# Autodesk Inventor assembly: КВ33.000.100 - Блок переключение передач
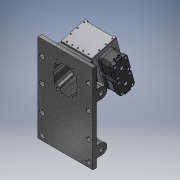
[picture p0: Inventor's stored thumbnail of the model, 180x180]
Saved by Autodesk Inventor 2019 (Build 230136000, 136)
## iProperties
Created: 2021-02-22
Part Number: КВ33.000.100 - Блок переключение передач
Material: Типовые
Document SubType Name: Assembly
Designer: Петров Иван
Author: Петров Иван
## Documents named in this file (12)
- E:\IVAN\Ivan_desktop\Kvantorium\Projects\tractor\design\КВ33.000.100 - Блок переключение передач.iam
- E:\IVAN\Ivan_desktop\Kvantorium\Projects\tractor\design\design_models\крышка КП.ipt
- E:\IVAN\Ivan_desktop\Kvantorium\Projects\tractor\design\КВ33.000.101 - Площадка крепежная.ipt
- E:\IVAN\Ivan_desktop\Kvantorium\Projects\tractor\design\КВ33.000.102 - Стенка толстая.ipt
- E:\IVAN\Ivan_desktop\Kvantorium\Projects\tractor\design\КВ33.000.103 - Стенка тонкая.ipt
- C:\Users\Петров Иван\Documents\Inventor\Content Center Files\R2019\en-US\GOST 9649-78\Washer 3 GOST 9649-78.ipt
- C:\Users\Петров Иван\Documents\Inventor\Content Center Files\R2019\en-US\Screw A2 GOST 17473-80\Screw A2.M2.5-6gx7 GOST 17473-80.ipt
- E:\IVAN\Ivan_desktop\Kvantorium\Projects\tractor\design\КВ33.000.104 - Крышка.ipt
- E:\IVAN\Ivan_desktop\Kvantorium\Projects\tractor\design\standart_components\Вал.ipt
- E:\IVAN\Ivan_desktop\Kvantorium\Projects\tractor\design\standart_components\Подшипник 626Z.ipt
- E:\IVAN\Ivan_desktop\Kvantorium\Projects\tractor\design\КВ33.000.105 - Заслонка.ipt
- E:\IVAN\Ivan_desktop\Kvantorium\Projects\tractor\design\standart_components\nema 17 motor.ipt
## Components (70 placed, 11 different names)
1. крышка КП:1 — Mate:1, Mate:8, Mate:9
2. КВ33.000.101 - Площадка крепежная:1 — Mate:1, Mate:3, Angle:1, Mate:4, Mate:6, Mate:8, Mate:9, Mate:21, Mate:27, Mate:28
3. КВ33.000.102 - Стенка толстая:1 — Mate:3, Angle:1, Insert:6, Insert:7, Insert:8, Insert:9, Insert:10, Mate:14, Mate:15, Mate:16, Mate:17, Mate:20, Mate:23, Angle:2, Angle:3, Mate:25, Mate:26
4. КВ33.000.102 - Стенка толстая:2 — Mate:4, Insert:1, Insert:2, Insert:3, Insert:4, Insert:5, Flush:4, Mate:10, Mate:11, Mate:12, Mate:13, Flush:5, Mate:28
5. КВ33.000.103 - Стенка тонкая:2 — Mate:6, Insert:22, Insert:23, Insert:24, Insert:25, Insert:26, Insert:27, Insert:28, Insert:29, Insert:30, Insert:31, Insert:32, Mate:21
6. КВ33.000.104 - Крышка:1 — Flush:4
7. Подшипник 626Z:1 — Mate:10, Mate:11, Mate:18
8. Подшипник 626Z:2 — Mate:14, Mate:15
9. Подшипник 626Z:3 — Mate:16, Mate:17
10. Подшипник 626Z:4 — Mate:12, Mate:13, Mate:19
11. Вал:1 — Mate:18, Flush:5, Flush:6, Mate:24
12. Вал:2 — Mate:19, Flush:6, Mate:22
13. КВ33.000.105 - Заслонка:1 — Mate:20
14. nema 17 motor:1 — Mate:22, Mate:23, Angle:2
15. nema 17 motor:2 — Mate:24, Angle:3
16. КВ33.000.103 - Стенка тонкая:3 — Mate:25, Mate:26, Mate:27
17. Washer GOST 9649-78 3:1 — Insert:1, Insert:49
18. Washer GOST 9649-78 3:2 — Insert:2, Insert:50
19. Washer GOST 9649-78 3:3 — Insert:3, Insert:51
20. Washer GOST 9649-78 3:4 — Insert:4, Insert:52
21. Washer GOST 9649-78 3:5 — Insert:5, Insert:53
22. Washer GOST 9649-78 3:6 — Insert:6, Insert:33
23. Washer GOST 9649-78 3:7 — Insert:7, Insert:34
24. Washer GOST 9649-78 3:8 — Insert:8, Insert:35
25. Washer GOST 9649-78 3:9 — Insert:9, Insert:36
26. Washer GOST 9649-78 3:10 — Insert:10, Insert:37
27. Washer GOST 9649-78 3:11 — Insert:42
28. Washer GOST 9649-78 3:12 — Insert:40
29. Washer GOST 9649-78 3:13 — Insert:41
30. Washer GOST 9649-78 3:14 — Insert:39
31. Washer GOST 9649-78 3:15 — Insert:38
32. Washer GOST 9649-78 3:16 — Insert:45
33. Washer GOST 9649-78 3:17 — Insert:44
34. Washer GOST 9649-78 3:18 — Insert:43
35. Washer GOST 9649-78 3:19 — Insert:46
36. Washer GOST 9649-78 3:20 — Insert:47
37. Washer GOST 9649-78 3:21 — Insert:48
38. Washer GOST 9649-78 3:22 — Insert:22
39. Washer GOST 9649-78 3:23 — Insert:23
40. Washer GOST 9649-78 3:24 — Insert:24
41. Washer GOST 9649-78 3:25 — Insert:25
42. Washer GOST 9649-78 3:26 — Insert:26
43. Washer GOST 9649-78 3:27 — Insert:27
44. Washer GOST 9649-78 3:28 — Insert:28
45. Washer GOST 9649-78 3:29 — Insert:29
46. Washer GOST 9649-78 3:30 — Insert:30, Insert:54
47. Washer GOST 9649-78 3:31 — Insert:31
48. Washer GOST 9649-78 3:32 — Insert:32
49. Screw A2 GOST 17473-80 M2.5-6gx7:1 — Insert:33
50. Screw A2 GOST 17473-80 M2.5-6gx7:2 — Insert:34
51. Screw A2 GOST 17473-80 M2.5-6gx7:3 — Insert:35
52. Screw A2 GOST 17473-80 M2.5-6gx7:4 — Insert:36
53. Screw A2 GOST 17473-80 M2.5-6gx7:5 — Insert:37
54. Screw A2 GOST 17473-80 M2.5-6gx7:6 — Insert:38
55. Screw A2 GOST 17473-80 M2.5-6gx7:7 — Insert:39
56. Screw A2 GOST 17473-80 M2.5-6gx7:8 — Insert:40
57. Screw A2 GOST 17473-80 M2.5-6gx7:9 — Insert:41
58. Screw A2 GOST 17473-80 M2.5-6gx7:10 — Insert:42
59. Screw A2 GOST 17473-80 M2.5-6gx7:11 — Insert:43
60. Screw A2 GOST 17473-80 M2.5-6gx7:12 — Insert:44
61. Screw A2 GOST 17473-80 M2.5-6gx7:13 — Insert:45
62. Screw A2 GOST 17473-80 M2.5-6gx7:14 — Insert:46
63. Screw A2 GOST 17473-80 M2.5-6gx7:15 — Insert:47
64. Screw A2 GOST 17473-80 M2.5-6gx7:16 — Insert:48
65. Screw A2 GOST 17473-80 M2.5-6gx7:17 — Insert:49
66. Screw A2 GOST 17473-80 M2.5-6gx7:18 — Insert:50
67. Screw A2 GOST 17473-80 M2.5-6gx7:19 — Insert:51
68. Screw A2 GOST 17473-80 M2.5-6gx7:20 — Insert:52
69. Screw A2 GOST 17473-80 M2.5-6gx7:21 — Insert:53
70. Screw A2 GOST 17473-80 M2.5-6gx7:22 — Insert:54
## Relationships (74: Insert 43, Mate 25, Angle 3, Flush 3)
- Mate:1: крышка КП:1 ↔ КВ33.000.101 - Площадка крепежная:1
- Mate:3: КВ33.000.101 - Площадка крепежная:1 ↔ КВ33.000.102 - Стенка толстая:1
- Angle:1 (0 deg): КВ33.000.101 - Площадка крепежная:1 ↔ КВ33.000.102 - Стенка толстая:1
- Mate:4: КВ33.000.101 - Площадка крепежная:1 ↔ КВ33.000.102 - Стенка толстая:2
- Mate:6: КВ33.000.101 - Площадка крепежная:1 ↔ КВ33.000.103 - Стенка тонкая:2
- Insert:1: КВ33.000.102 - Стенка толстая:2 ↔ Washer GOST 9649-78 3:1
- Insert:2: КВ33.000.102 - Стенка толстая:2 ↔ Washer GOST 9649-78 3:2
- Insert:3: КВ33.000.102 - Стенка толстая:2 ↔ Washer GOST 9649-78 3:3
- Insert:4: КВ33.000.102 - Стенка толстая:2 ↔ Washer GOST 9649-78 3:4
- Insert:5: КВ33.000.102 - Стенка толстая:2 ↔ Washer GOST 9649-78 3:5
- Insert:6: КВ33.000.102 - Стенка толстая:1 ↔ Washer GOST 9649-78 3:6
- Insert:7: КВ33.000.102 - Стенка толстая:1 ↔ Washer GOST 9649-78 3:7
- Insert:8: КВ33.000.102 - Стенка толстая:1 ↔ Washer GOST 9649-78 3:8
- Insert:9: КВ33.000.102 - Стенка толстая:1 ↔ Washer GOST 9649-78 3:9
- Insert:10: КВ33.000.102 - Стенка толстая:1 ↔ Washer GOST 9649-78 3:10
- Insert:22: КВ33.000.103 - Стенка тонкая:2 ↔ Washer GOST 9649-78 3:22
- Insert:23: КВ33.000.103 - Стенка тонкая:2 ↔ Washer GOST 9649-78 3:23
- Insert:24: КВ33.000.103 - Стенка тонкая:2 ↔ Washer GOST 9649-78 3:24
- Insert:25: КВ33.000.103 - Стенка тонкая:2 ↔ Washer GOST 9649-78 3:25
- Insert:26: КВ33.000.103 - Стенка тонкая:2 ↔ Washer GOST 9649-78 3:26
- Insert:27: КВ33.000.103 - Стенка тонкая:2 ↔ Washer GOST 9649-78 3:27
- Insert:28: КВ33.000.103 - Стенка тонкая:2 ↔ Washer GOST 9649-78 3:28
- Insert:29: КВ33.000.103 - Стенка тонкая:2 ↔ Washer GOST 9649-78 3:29
- Insert:30: КВ33.000.103 - Стенка тонкая:2 ↔ Washer GOST 9649-78 3:30
- Insert:31: КВ33.000.103 - Стенка тонкая:2 ↔ Washer GOST 9649-78 3:31
- Insert:32: КВ33.000.103 - Стенка тонкая:2 ↔ Washer GOST 9649-78 3:32
- Insert:33: Washer GOST 9649-78 3:6 ↔ Screw A2 GOST 17473-80 M2.5-6gx7:1
- Insert:34: Washer GOST 9649-78 3:7 ↔ Screw A2 GOST 17473-80 M2.5-6gx7:2
- Insert:35: Washer GOST 9649-78 3:8 ↔ Screw A2 GOST 17473-80 M2.5-6gx7:3
- Insert:36: Washer GOST 9649-78 3:9 ↔ Screw A2 GOST 17473-80 M2.5-6gx7:4
- Insert:37: Washer GOST 9649-78 3:10 ↔ Screw A2 GOST 17473-80 M2.5-6gx7:5
- Insert:38: Washer GOST 9649-78 3:15 ↔ Screw A2 GOST 17473-80 M2.5-6gx7:6
- Insert:39: Washer GOST 9649-78 3:14 ↔ Screw A2 GOST 17473-80 M2.5-6gx7:7
- Insert:40: Washer GOST 9649-78 3:12 ↔ Screw A2 GOST 17473-80 M2.5-6gx7:8
- Insert:41: Washer GOST 9649-78 3:13 ↔ Screw A2 GOST 17473-80 M2.5-6gx7:9
- Insert:42: Washer GOST 9649-78 3:11 ↔ Screw A2 GOST 17473-80 M2.5-6gx7:10
- Insert:43: Washer GOST 9649-78 3:18 ↔ Screw A2 GOST 17473-80 M2.5-6gx7:11
- Insert:44: Washer GOST 9649-78 3:17 ↔ Screw A2 GOST 17473-80 M2.5-6gx7:12
- Insert:45: Washer GOST 9649-78 3:16 ↔ Screw A2 GOST 17473-80 M2.5-6gx7:13
- Insert:46: Washer GOST 9649-78 3:19 ↔ Screw A2 GOST 17473-80 M2.5-6gx7:14
- Insert:47: Washer GOST 9649-78 3:20 ↔ Screw A2 GOST 17473-80 M2.5-6gx7:15
- Insert:48: Washer GOST 9649-78 3:21 ↔ Screw A2 GOST 17473-80 M2.5-6gx7:16
- Insert:49: Washer GOST 9649-78 3:1 ↔ Screw A2 GOST 17473-80 M2.5-6gx7:17
- Insert:50: Washer GOST 9649-78 3:2 ↔ Screw A2 GOST 17473-80 M2.5-6gx7:18
- Insert:51: Washer GOST 9649-78 3:3 ↔ Screw A2 GOST 17473-80 M2.5-6gx7:19
- Insert:52: Washer GOST 9649-78 3:4 ↔ Screw A2 GOST 17473-80 M2.5-6gx7:20
- Insert:53: Washer GOST 9649-78 3:5 ↔ Screw A2 GOST 17473-80 M2.5-6gx7:21
- Insert:54: Washer GOST 9649-78 3:30 ↔ Screw A2 GOST 17473-80 M2.5-6gx7:22
- Flush:4: КВ33.000.102 - Стенка толстая:2 ↔ КВ33.000.104 - Крышка:1
- Mate:8: крышка КП:1 ↔ КВ33.000.101 - Площадка крепежная:1
- Mate:9: крышка КП:1 ↔ КВ33.000.101 - Площадка крепежная:1
- Mate:10: КВ33.000.102 - Стенка толстая:2 ↔ Подшипник 626Z:1
- Mate:11: КВ33.000.102 - Стенка толстая:2 ↔ Подшипник 626Z:1
- Mate:12: КВ33.000.102 - Стенка толстая:2 ↔ Подшипник 626Z:4
- Mate:13: КВ33.000.102 - Стенка толстая:2 ↔ Подшипник 626Z:4
- Mate:14: КВ33.000.102 - Стенка толстая:1 ↔ Подшипник 626Z:2
- Mate:15: КВ33.000.102 - Стенка толстая:1 ↔ Подшипник 626Z:2
- Mate:16: КВ33.000.102 - Стенка толстая:1 ↔ Подшипник 626Z:3
- Mate:17: КВ33.000.102 - Стенка толстая:1 ↔ Подшипник 626Z:3
- Mate:18: Подшипник 626Z:1 ↔ Вал:1
- Flush:5 (-7.5 mm): КВ33.000.102 - Стенка толстая:2 ↔ Вал:1
- Mate:19: Подшипник 626Z:4 ↔ Вал:2
- Flush:6: Вал:1 ↔ Вал:2
- Mate:20: КВ33.000.102 - Стенка толстая:1 ↔ КВ33.000.105 - Заслонка:1
- Mate:21: КВ33.000.101 - Площадка крепежная:1 ↔ КВ33.000.103 - Стенка тонкая:2
- Mate:22: Вал:2 ↔ nema 17 motor:1
- Mate:23 (5 mm): КВ33.000.102 - Стенка толстая:1 ↔ nema 17 motor:1
- Angle:2 (0 deg): КВ33.000.102 - Стенка толстая:1 ↔ nema 17 motor:1
- Mate:24: Вал:1 ↔ nema 17 motor:2
- Angle:3 (0 deg): КВ33.000.102 - Стенка толстая:1 ↔ nema 17 motor:2
- Mate:25: КВ33.000.102 - Стенка толстая:1 ↔ КВ33.000.103 - Стенка тонкая:3
- Mate:26: КВ33.000.102 - Стенка толстая:1 ↔ КВ33.000.103 - Стенка тонкая:3
- Mate:27: КВ33.000.101 - Площадка крепежная:1 ↔ КВ33.000.103 - Стенка тонкая:3
- Mate:28: КВ33.000.101 - Площадка крепежная:1 ↔ КВ33.000.102 - Стенка толстая:2
